# Autodesk Inventor assembly: RCUv2-1
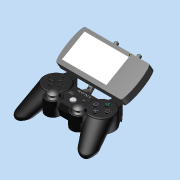
[picture p0: Inventor's stored thumbnail of the model, 180x180]
Saved by Autodesk Inventor 2011 SP1 (Build 150282100, 282)
## iProperties
Created: 2011-08-14
Part Number: RCUv2-1
Document SubType Name: Assembly
Designer: dgitz
Author: dgitz
## Documents named in this file (4)
- C:\Dropbox\ICARUS\Remote Control Unit (RCU)\RCU v2\Design\RCUv2-1.iam
- C:\Dropbox\ICARUS\Remote Control Unit (RCU)\RCU v2\Design\Library\PS2 Controller-Wireless.iam
- C:\Dropbox\ICARUS\Remote Control Unit (RCU)\RCU v2\Design\Library\SpringSamsungGalaxySAssy.iam
- C:\Dropbox\ICARUS\Remote Control Unit (RCU)\RCU v2\Design\Library\XBeeAntennaAssy.iam
## Components (4 placed, 3 different names)
1. PS2 Controller-Wireless:1 [sub-assembly] — Flush:1, Mate:1, Angle:1, Mate:2, Mate:3, Mate:4
2. SpringSamsungGalaxySAssy:1 [sub-assembly] — Angle:1, Mate:2
3. XBeeAntennaAssy:1 [sub-assembly] — Mate:3, Angle:2
4. XBeeAntennaAssy:2 [sub-assembly] — Mate:4, Angle:2
## Relationships (7: Mate 4, Angle 2, Flush 1)
- Flush:1: PS2 Controller-Wireless:1
- Mate:1: PS2 Controller-Wireless:1
- Angle:1 (30 deg): PS2 Controller-Wireless:1 ↔ SpringSamsungGalaxySAssy:1
- Mate:2: PS2 Controller-Wireless:1 ↔ SpringSamsungGalaxySAssy:1
- Mate:3: PS2 Controller-Wireless:1 ↔ XBeeAntennaAssy:1
- Mate:4: PS2 Controller-Wireless:1 ↔ XBeeAntennaAssy:2
- Angle:2 (0 deg): XBeeAntennaAssy:1 ↔ XBeeAntennaAssy:2
